# Autodesk Inventor assembly: Mesa_Tubo
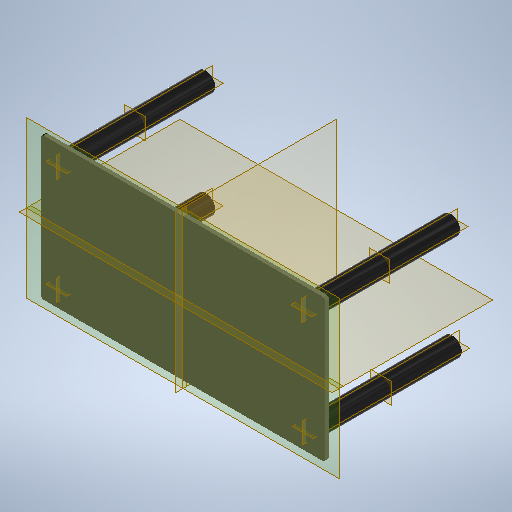
[picture p0: Inventor's stored thumbnail of the model, 512x512]
Saved by Autodesk Inventor 2025.2 (Build 292293000, 293)
## iProperties
Created: 2025-03-28
Part Number: Mesa_Tubo
Document SubType Name: Assembly
Designer: ishad
Author: ishad
## Documents named in this file (3)
- C:\Users\ishad\Documents\Inventor\Sessao_6\Mesa_Tubo.iam
- C:\Users\ishad\Documents\Inventor\Sessao_6\Mesa_001_0002.ipt
- C:\Users\ishad\Documents\Inventor\Sessao_6\Tubo_0001.ipt
## Components (5 placed, 2 different names)
1. Mesa_001_0002:1 — Flush:1, Mate:1, Mate:2, Mate:3, Mate:4
2. Tubo_0001:1 — Mate:4, Flush:2, Flush:3, Flush:4, Flush:5, Flush:7, Flush:9, Flush:11, Symmetry:1, Symmetry:2
3. Tubo_0001:2 — Flush:5, Flush:8, Flush:10, Symmetry:1, Symmetry:2
4. Tubo_0001:4 — Flush:4, Flush:9, Flush:10
5. Tubo_0001:6 — Flush:7, Flush:8, Flush:11
## Relationships (16: Flush 10, Mate 4, Symmetry 2)
- Flush:1: Mesa_001_0002:1
- Mate:1: Mesa_001_0002:1
- Mate:2: Mesa_001_0002:1
- Mate:3: Mesa_001_0002:1
- Mate:4: Mesa_001_0002:1 ↔ Tubo_0001:1
- Flush:2 (280 mm): Tubo_0001:1
- Flush:3 (650 mm): Tubo_0001:1
- Flush:4 (-0.117 mm): Tubo_0001:1 ↔ Tubo_0001:4
- Flush:5 (8.799 mm): Tubo_0001:1 ↔ Tubo_0001:2
- Flush:7: Tubo_0001:1 ↔ Tubo_0001:6
- Flush:8: Tubo_0001:2 ↔ Tubo_0001:6
- Flush:9: Tubo_0001:1 ↔ Tubo_0001:4
- Flush:10: Tubo_0001:2 ↔ Tubo_0001:4
- Flush:11: Tubo_0001:1 ↔ Tubo_0001:6
- Symmetry:1: Tubo_0001:1 ↔ Tubo_0001:2
- Symmetry:2: Tubo_0001:1 ↔ Tubo_0001:2
